# Autodesk Inventor assembly: CIM Motor
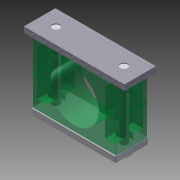
[picture p0: Inventor's stored thumbnail of the model, 180x180]
Saved by Autodesk Inventor 2013 (Build 170138000, 138)
## iProperties
Created: 2013-01-18
Part Number: CIM Motor
Document SubType Name: Assembly
Designer: Naphat
Author: Naphat
## Documents named in this file (5)
- C:\Users\carneeki\Desktop\Kiwi Robot\Imported Components\Motors\CIM Mount\CIM Mount.iam
- C:\Users\carneeki\Desktop\Kiwi Robot\Imported Components\Motors\CIM Mount\CIM Mount Half.ipt
- C:\Users\carneeki\Desktop\Kiwi Robot\Imported Components\Motors\CIM Mount\CIM Mount Top.ipt
- C:\Users\carneeki\Desktop\Kiwi Robot\Imported Components\Motors\CIM Mount\CIM Mount Base.ipt
- C:\Users\carneeki\Desktop\Kiwi Robot\Imported Components\Motors\CIM Mount\CIM Mount Bolt.ipt
## Components (6 placed, 4 different names)
1. CIM Mount Half:1 — Mate:1, Mate:2, Mate:3, Mate:4, Mate:15, Mate:16, Mate:17
2. CIM Mount Half:2 — Mate:1, Mate:2, Mate:3, Mate:4, Mate:10, Mate:12, Mate:13, Mate:14
3. CIM Mount Top:1 — Mate:10, Mate:12, Mate:13, Mate:14, Mate:18, Mate:19, Mate:20, Mate:21
4. CIM Mount Base:1 — Mate:15, Mate:16, Mate:17
5. CIM Mount Bolt:1 — Mate:18, Mate:19
6. CIM Mount Bolt:2 — Mate:20, Mate:21
## Relationships (15: Mate 15)
- Mate:1: CIM Mount Half:1 ↔ CIM Mount Half:2
- Mate:2: CIM Mount Half:1 ↔ CIM Mount Half:2
- Mate:3: CIM Mount Half:1 ↔ CIM Mount Half:2
- Mate:4: CIM Mount Half:1 ↔ CIM Mount Half:2
- Mate:10: CIM Mount Half:2 ↔ CIM Mount Top:1
- Mate:12: CIM Mount Half:2 ↔ CIM Mount Top:1
- Mate:13: CIM Mount Half:2 ↔ CIM Mount Top:1
- Mate:14: CIM Mount Half:2 ↔ CIM Mount Top:1
- Mate:15: CIM Mount Half:1 ↔ CIM Mount Base:1
- Mate:16: CIM Mount Half:1 ↔ CIM Mount Base:1
- Mate:17: CIM Mount Half:1 ↔ CIM Mount Base:1
- Mate:18: CIM Mount Top:1 ↔ CIM Mount Bolt:1
- Mate:19: CIM Mount Top:1 ↔ CIM Mount Bolt:1
- Mate:20: CIM Mount Top:1 ↔ CIM Mount Bolt:2
- Mate:21: CIM Mount Top:1 ↔ CIM Mount Bolt:2
